# Autodesk Inventor assembly: Сборка_Концепт_новый
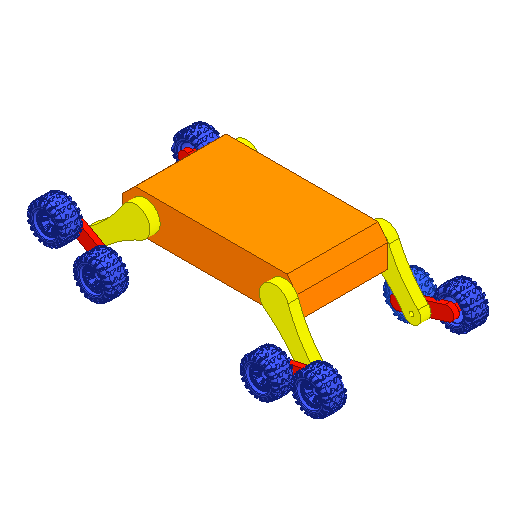
[picture p0: Inventor's stored thumbnail of the model, 512x512]
Saved by Autodesk Inventor 2026 (Build 300175000, 175)
## iProperties
Created: 2026-04-19
Part Number: Сборка_Концепт_новый
Document SubType Name: Assembly
Designer: Artem Sannikov
Author: Artem Sannikov
## Documents named in this file (16)
- C:\Users\Artem Sannikov\Desktop\Robo-Forester\3D\Сборка_Концепт_новый.iam
- C:\Users\Artem Sannikov\Desktop\Robo-Forester\3D\Колено.ipt
- C:\Users\Artem Sannikov\Desktop\Robo-Forester\3D\Нога.ipt
- C:\Users\Artem Sannikov\Desktop\Robo-Forester\3D\Тело.ipt
- C:\Users\Artem Sannikov\Desktop\Robo-Forester\3D\Колесо_Новое.ipt
- C:\Users\Artem Sannikov\Desktop\Robo-Forester\3D\Ось_Схематично.ipt
- C:\Users\Artem Sannikov\Desktop\Robo-Forester\3D\Ось_Схематично_MIR.ipt
- C:\Users\Artem Sannikov\Desktop\Robo-Forester\3D\Рабочая область.ipt
- C:\Users\Artem Sannikov\Desktop\Robo-Forester\3D\РабОбласть2.ipt
- C:\Users\Artem Sannikov\Desktop\Robo-Forester\3D\Ось_Схематично_MIR1.ipt
- C:\Users\Artem Sannikov\Desktop\Robo-Forester\3D\РабЗона3.ipt
- C:\Users\Artem Sannikov\Desktop\Robo-Forester\3D\Диск.ipt
- C:\Users\Artem Sannikov\Desktop\Robo-Forester\3D\Гайка.ipt
- C:\Users\Artem Sannikov\Desktop\Robo-Forester\3D\Винт.ipt
- C:\Users\Artem Sannikov\Desktop\Robo-Forester\3D\Моторчик_Замка.ipt
- C:\Users\Artem Sannikov\Desktop\Robo-Forester\3D\Рейка.ipt
## Components (44 placed, 15 different names)
1. Колено:1 — Совмещение:3, Совмещение:18, Совмещение:19, Совмещение:20, Совмещение:21, Совмещение:22, Совмещение:24, Совмещение:52
2. Нога:1 — Заподлицо:3, Совмещение:3, Совмещение:4, Совмещение:18, Совмещение:39, Совмещение:40, Совмещение:51, Совмещение:53, Совмещение:54, Заподлицо:13, Совмещение:75
3. Тело:1 — Заподлицо:3, Совмещение:4, Совмещение:5, Заподлицо:4, Заподлицо:5, Совмещение:6, Совмещение:7, Совмещение:8, Совмещение:9, Совмещение:10, Совмещение:11, Заподлицо:6, Совмещение:56
4. Нога:2 — Совмещение:6, Совмещение:7, Совмещение:12, Совмещение:13, Совмещение:37, Совмещение:38, Заподлицо:9, Заподлицо:10
5. Нога:3 — Совмещение:10, Совмещение:11, Совмещение:16, Совмещение:17, Совмещение:60, Совмещение:63, Совмещение:70
6. Нога:4 — Совмещение:8, Совмещение:9, Совмещение:14, Совмещение:15, Совмещение:59, Совмещение:66, Совмещение:74
7. Колено:2 — Совмещение:12, Совмещение:13, Совмещение:23, Совмещение:25, Совмещение:26, Совмещение:27, Заподлицо:7, Заподлицо:8, Совмещение:50
8. Колено:3 — Совмещение:14, Совмещение:15, Совмещение:31, Совмещение:32, Совмещение:33, Совмещение:34, Совмещение:73
9. Колено:4 — Совмещение:16, Совмещение:17, Совмещение:28, Совмещение:29, Совмещение:30, Совмещение:35, Совмещение:36, Совмещение:69
10. Колесо_Новое:1 — Совмещение:19, Совмещение:20, Совмещение:24, Совмещение:45, Совмещение:46
11. Колесо_Новое:2 — Совмещение:21, Совмещение:22, Совмещение:47, Совмещение:48
12. Колесо_Новое:3 — Совмещение:23, Совмещение:25, Совмещение:41, Совмещение:42
13. Колесо_Новое:4 — Совмещение:26, Совмещение:27, Совмещение:43, Совмещение:44
14. Колесо_Новое:5 — Совмещение:31, Совмещение:32, Совмещение:64, Совмещение:72
15. Колесо_Новое:6 — Совмещение:33, Совмещение:34, Совмещение:65, Совмещение:71
16. Колесо_Новое:7 — Совмещение:30, Совмещение:35, Совмещение:36, Совмещение:62, Совмещение:68
17. Колесо_Новое:8 — Совмещение:28, Совмещение:29, Совмещение:61, Совмещение:67
18. Ось_Схематично:1 — Совмещение:37, Совмещение:38
19. Ось_Схематично:2 — Совмещение:39, Совмещение:40, Совмещение:55, Совмещение:57
20. Ось_Схематично:3 — Совмещение:41, Совмещение:42
21. Ось_Схематично:4 — Совмещение:43, Совмещение:44
22. Ось_Схематично:5 — Совмещение:45, Совмещение:46
23. Ось_Схематично:6 — Совмещение:47, Совмещение:48
24. Ось_Схематично_MIR:1 — Совмещение:59, Совмещение:74
25. Ось_Схематично_MIR:2 — Совмещение:60, Совмещение:70
26. Ось_Схематично_MIR:3 — Совмещение:64, Совмещение:72
27. Ось_Схематично_MIR:4 — Совмещение:65, Совмещение:71
28. Ось_Схематично_MIR:5 — Совмещение:61, Совмещение:67
29. Ось_Схематично_MIR:6 — Совмещение:62, Совмещение:68
30. Рабочая область:1 — Заподлицо:7, Заподлицо:8, Совмещение:49
31. РабОбласть2:1 — Заподлицо:9, Заподлицо:10, Заподлицо:11, Заподлицо:12
32. Ось_Схематично:7 — Совмещение:49, Совмещение:50
33. Ось_Схематично:8 — Совмещение:51, Совмещение:52
34. Ось_Схематично_MIR1:1 — Совмещение:66, Совмещение:73
35. Ось_Схематично_MIR1:2 — Совмещение:63, Совмещение:69
36. РабЗона3:1 — Заподлицо:11, Заподлицо:12
37. Рабочая область:2 — Совмещение:53, Совмещение:54
38. РабОбласть2:2 — Совмещение:55, Совмещение:56, Совмещение:58
39. РабЗона3:2 — Совмещение:57, Совмещение:58
40. Диск:1 — Заподлицо:13, Совмещение:75, Заподлицо:14, Заподлицо:15
41. Гайка:1 — Заподлицо:14, Заподлицо:15, Заподлицо:16, Заподлицо:18, Заподлицо:19
42. Винт:1 — Заподлицо:16, Заподлицо:17
43. Моторчик_Замка:1 — Заподлицо:17
44. Рейка:1 — Заподлицо:18, Заподлицо:19
## Relationships (90: Mate 73, Flush 17)
- Заподлицо:3 [Flush]: Нога:1 ↔ Тело:1
- Совмещение:3 [Mate]: Колено:1 ↔ Нога:1
- Совмещение:4 [Mate]: Нога:1 ↔ Тело:1
- Совмещение:5 [Mate]: Тело:1
- Заподлицо:4 [Flush]: Тело:1
- Заподлицо:5 [Flush]: Тело:1
- Совмещение:6 [Mate]: Тело:1 ↔ Нога:2
- Совмещение:7 [Mate]: Тело:1 ↔ Нога:2
- Совмещение:8 [Mate]: Тело:1 ↔ Нога:4
- Совмещение:9 [Mate]: Тело:1 ↔ Нога:4
- Совмещение:10 [Mate]: Тело:1 ↔ Нога:3
- Совмещение:11 [Mate]: Тело:1 ↔ Нога:3
- Совмещение:12 [Mate]: Нога:2 ↔ Колено:2
- Совмещение:13 [Mate]: Нога:2 ↔ Колено:2
- Совмещение:14 [Mate]: Нога:4 ↔ Колено:3
- Совмещение:15 [Mate]: Нога:4 ↔ Колено:3
- Совмещение:16 [Mate]: Нога:3 ↔ Колено:4
- Совмещение:17 [Mate]: Нога:3 ↔ Колено:4
- Совмещение:18 [Mate]: Колено:1 ↔ Нога:1
- Совмещение:19 [Mate]: Колено:1 ↔ Колесо_Новое:1
- Совмещение:20 [Mate]: Колено:1 ↔ Колесо_Новое:1
- Совмещение:21 [Mate]: Колено:1 ↔ Колесо_Новое:2
- Совмещение:22 [Mate]: Колено:1 ↔ Колесо_Новое:2
- Совмещение:23 [Mate]: Колено:2 ↔ Колесо_Новое:3
- Совмещение:24 [Mate]: Колено:1 ↔ Колесо_Новое:1
- Совмещение:25 [Mate]: Колено:2 ↔ Колесо_Новое:3
- Совмещение:26 [Mate]: Колено:2 ↔ Колесо_Новое:4
- Совмещение:27 [Mate]: Колено:2 ↔ Колесо_Новое:4
- Совмещение:28 [Mate]: Колено:4 ↔ Колесо_Новое:8
- Совмещение:29 [Mate]: Колено:4 ↔ Колесо_Новое:8
- Совмещение:30 [Mate]: Колено:4 ↔ Колесо_Новое:7
- Совмещение:31 [Mate]: Колено:3 ↔ Колесо_Новое:5
- Совмещение:32 [Mate]: Колено:3 ↔ Колесо_Новое:5
- Совмещение:33 [Mate]: Колено:3 ↔ Колесо_Новое:6
- Совмещение:34 [Mate]: Колено:3 ↔ Колесо_Новое:6
- Совмещение:35 [Mate]: Колено:4 ↔ Колесо_Новое:7
- Совмещение:36 [Mate]: Колено:4 ↔ Колесо_Новое:7
- Совмещение:37 [Mate]: Нога:2 ↔ Ось_Схематично:1
- Совмещение:38 [Mate]: Нога:2 ↔ Ось_Схематично:1
- Совмещение:39 [Mate]: Нога:1 ↔ Ось_Схематично:2
- Совмещение:40 [Mate]: Нога:1 ↔ Ось_Схематично:2
- Совмещение:41 [Mate]: Колесо_Новое:3 ↔ Ось_Схематично:3
- Совмещение:42 [Mate]: Колесо_Новое:3 ↔ Ось_Схематично:3
- Совмещение:43 [Mate]: Колесо_Новое:4 ↔ Ось_Схематично:4
- Совмещение:44 [Mate]: Колесо_Новое:4 ↔ Ось_Схематично:4
- Совмещение:45 [Mate]: Колесо_Новое:1 ↔ Ось_Схематично:5
- Совмещение:46 [Mate]: Колесо_Новое:1 ↔ Ось_Схематично:5
- Совмещение:47 [Mate]: Колесо_Новое:2 ↔ Ось_Схематично:6
- Совмещение:48 [Mate]: Колесо_Новое:2 ↔ Ось_Схематично:6
- Заподлицо:6 [Flush] (-200 mm): Тело:1
- Заподлицо:7 [Flush]: Колено:2 ↔ Рабочая область:1
- Заподлицо:8 [Flush]: Колено:2 ↔ Рабочая область:1
- Заподлицо:9 [Flush]: Нога:2 ↔ РабОбласть2:1
- Заподлицо:10 [Flush]: Нога:2 ↔ РабОбласть2:1
- Совмещение:49 [Mate]: Рабочая область:1 ↔ Ось_Схематично:7
- Совмещение:50 [Mate]: Колено:2 ↔ Ось_Схематично:7
- Совмещение:51 [Mate]: Нога:1 ↔ Ось_Схематично:8
- Совмещение:52 [Mate]: Колено:1 ↔ Ось_Схематично:8
- Заподлицо:11 [Flush]: РабОбласть2:1 ↔ РабЗона3:1
- Заподлицо:12 [Flush]: РабОбласть2:1 ↔ РабЗона3:1
- Совмещение:53 [Mate]: Нога:1 ↔ Рабочая область:2
- Совмещение:54 [Mate]: Нога:1 ↔ Рабочая область:2
- Совмещение:55 [Mate]: Ось_Схематично:2 ↔ РабОбласть2:2
- Совмещение:56 [Mate]: Тело:1 ↔ РабОбласть2:2
- Совмещение:57 [Mate]: Ось_Схематично:2 ↔ РабЗона3:2
- Совмещение:58 [Mate]: РабОбласть2:2 ↔ РабЗона3:2
- Совмещение:59 [Mate]: Нога:4 ↔ Ось_Схематично_MIR:1
- Совмещение:60 [Mate]: Нога:3 ↔ Ось_Схематично_MIR:2
- Совмещение:61 [Mate]: Колесо_Новое:8 ↔ Ось_Схематично_MIR:5
- Совмещение:62 [Mate]: Колесо_Новое:7 ↔ Ось_Схематично_MIR:6
- Совмещение:63 [Mate]: Нога:3 ↔ Ось_Схематично_MIR1:2
- Совмещение:64 [Mate]: Колесо_Новое:5 ↔ Ось_Схематично_MIR:3
- Совмещение:65 [Mate]: Колесо_Новое:6 ↔ Ось_Схематично_MIR:4
- Совмещение:66 [Mate]: Нога:4 ↔ Ось_Схематично_MIR1:1
- Совмещение:67 [Mate]: Колесо_Новое:8 ↔ Ось_Схематично_MIR:5
- Совмещение:68 [Mate]: Колесо_Новое:7 ↔ Ось_Схематично_MIR:6
- Совмещение:69 [Mate]: Колено:4 ↔ Ось_Схематично_MIR1:2
- Совмещение:70 [Mate]: Нога:3 ↔ Ось_Схематично_MIR:2
- Совмещение:71 [Mate]: Колесо_Новое:6 ↔ Ось_Схематично_MIR:4
- Совмещение:72 [Mate]: Колесо_Новое:5 ↔ Ось_Схематично_MIR:3
- Совмещение:73 [Mate]: Колено:3 ↔ Ось_Схематично_MIR1:1
- Совмещение:74 [Mate]: Нога:4 ↔ Ось_Схематично_MIR:1
- Заподлицо:13 [Flush]: Нога:1 ↔ Диск:1
- Совмещение:75 [Mate]: Нога:1 ↔ Диск:1
- Заподлицо:14 [Flush]: Диск:1 ↔ Гайка:1
- Заподлицо:15 [Flush]: Диск:1 ↔ Гайка:1
- Заподлицо:16 [Flush]: Гайка:1 ↔ Винт:1
- Заподлицо:17 [Flush]: Винт:1 ↔ Моторчик_Замка:1
- Заподлицо:18 [Flush]: Гайка:1 ↔ Рейка:1
- Заподлицо:19 [Flush]: Гайка:1 ↔ Рейка:1
